# Autodesk Inventor assembly: GT2Idler
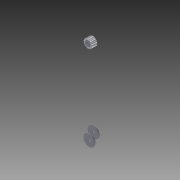
[picture p0: Inventor's stored thumbnail of the model, 180x180]
Saved by Autodesk Inventor 2015 SP1 (Build 190203100, 203)
## iProperties
Category: Hardware
Created: 2014-12-01
Part Number: GT2Idler
Document SubType Name: Assembly
Designer: Jack
Mass: 3.21077 g
Surface Area: 20.7758 cm^2
Volume: 0.962827 cm^3
Density: 3.33473 g/cm^3
Vendor: Misumi
Catalog Web Link: N/A
Author: Jack
Title: GT2 Toothed Idler
## Documents named in this file (5)
- C:\Users\Jack\ownCloud\Projects\CrossBot\InventorModel\Hardware\Belt\GT2Idler.iam
- C:\Users\Jack\ownCloud\Projects\CrossBot\InventorModel\Hardware\Belt\PulleyGT2x20Top.ipt
- C:\Users\Jack\ownCloud\Projects\CrossBot\InventorModel\Hardware\Bearing\BearingRadialBall\BearingRadialBall4x8x3.ipt
- C:\Users\Jack\ownCloud\Projects\CrossBot\InventorModel\Hardware\Wahsers\M3Washer.ipt
- C:\Users\Jack\ownCloud\Projects\CrossBot\InventorModel\Hardware\Wahsers\No6FenderWasher.ipt
## Components (7 placed, 4 different names)
1. PulleyGT2x20Top:1 — Mate:1, Mate:2, Flush:1, Mate:3, Flush:2
2. BearingRadialBall4x8x3:1 — Mate:1, Mate:3, Flush:2, Mate:5, Mate:6
3. BearingRadialBall4x8x3:2 — Mate:2, Flush:1, Mate:4, Mate:7
4. M3Washer:1 — Mate:5, Mate:6, Mate:9, Mate:10
5. M3Washer:2 — Mate:4, Mate:7, Mate:8, Mate:11
6. No6FenderWasher:1 — Mate:8, Mate:11
7. No6FenderWasher:2 — Mate:9, Mate:10
## Relationships (13: Mate 11, Flush 2)
- Mate:1: PulleyGT2x20Top:1 ↔ BearingRadialBall4x8x3:1
- Mate:2: PulleyGT2x20Top:1 ↔ BearingRadialBall4x8x3:2
- Flush:1: PulleyGT2x20Top:1 ↔ BearingRadialBall4x8x3:2
- Mate:3: PulleyGT2x20Top:1 ↔ BearingRadialBall4x8x3:1
- Flush:2: PulleyGT2x20Top:1 ↔ BearingRadialBall4x8x3:1
- Mate:4: BearingRadialBall4x8x3:2 ↔ M3Washer:2
- Mate:5: BearingRadialBall4x8x3:1 ↔ M3Washer:1
- Mate:6: BearingRadialBall4x8x3:1 ↔ M3Washer:1
- Mate:7: BearingRadialBall4x8x3:2 ↔ M3Washer:2
- Mate:8: M3Washer:2 ↔ No6FenderWasher:1
- Mate:9: M3Washer:1 ↔ No6FenderWasher:2
- Mate:10: M3Washer:1 ↔ No6FenderWasher:2
- Mate:11: M3Washer:2 ↔ No6FenderWasher:1
